# Autodesk Inventor assembly: 305-9
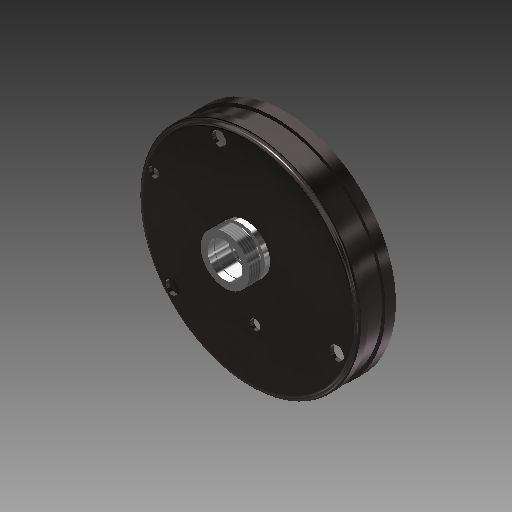
[picture p0: Inventor's stored thumbnail of the model, 512x512]
Saved by Autodesk Inventor 2019 (Build 230136000, 136)
## iProperties
Company: Autodesk Inc.
Created: 2012-01-27
Part Number: 305-9
Document SubType Name: Assembly
Designer: Autodesk Inc.
Mass: 45.6115 g
Surface Area: 115.977 cm^2
Volume: 5.71058 cm^3
Density: 7.9872 g/cm^3
Author: Inventor
## Documents named in this file (3)
- C:\TEMP\Fishing Rod\Workspaces\Back Side Cover Assembly.iam
- C:\TEMP\Fishing Rod\Workspaces\Bearing Housing.ipt
- C:\TEMP\Fishing Rod\Workspaces\Back Side Cover.ipt
## Components (2 placed, 2 different names)
1. Back Side Cover:1 — Insert:1
2. Bearing Housing:1 — Insert:1
## Relationships (1: Insert 1)
- Insert:1: Back Side Cover:1 ↔ Bearing Housing:1
